# Autodesk Inventor assembly: RailWheelSys
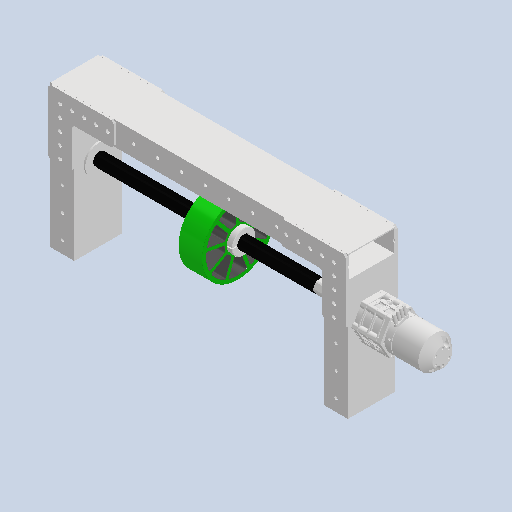
[picture p0: Inventor's stored thumbnail of the model, 512x512]
Saved by Autodesk Inventor 2022 (Build 260153000, 153)
## iProperties
Created: 2022-01-14
Part Number: RailWheelSys
Document SubType Name: Assembly
Designer: tagaz
Author: tagaz
## Documents named in this file (9)
- C:\Users\merky\OneDrive\Documents\t3-cad\CAD\2022 Parts\Index\RailWheelSys.iam
- C:\Users\merky\OneDrive\Documents\t3-cad\CAD\2022 Parts\Generic\RailSupp.ipt
- C:\Users\merky\OneDrive\Documents\t3-cad\CAD\Bearing  for THUNDER.ipt
- C:\Users\merky\OneDrive\Documents\t3-cad\CAD\2022 Parts\Generic\railThunder.ipt
- C:\Users\merky\OneDrive\Documents\t3-cad\CAD\2022 Parts\Generic\3in Compliance wheel.ipt
- C:\Users\merky\OneDrive\Documents\t3-cad\CAD\Hex Shaft Collar.ipt
- C:\Users\merky\OneDrive\Documents\t3-cad\CAD\2022 Parts\Generic\RailSupp2.ipt
- C:\Users\merky\OneDrive\Documents\t3-cad\CAD\Generic and Stock\VersaGusset 90o.ipt
- C:\Users\merky\OneDrive\Documents\t3-cad\CAD\Generic and Stock\RevMotorParts\Neo550Assembly.iam
## Components (15 placed, 8 different names)
1. RailSupp:1 — Mate:1, Flush:1, Flush:2, Insert:1, Insert:2, Mate:6, Flush:5, Mate:15, Flush:6, Flush:8, Flush:13
2. RailSupp:2 — Mate:1, Flush:1, Flush:2, Flush:10, Flush:12, Insert:3, Mate:21, Mate:22
3. Bearing  for THUNDER:1 — Insert:1
4. Bearing  for THUNDER:2 — Insert:2, Mate:2, Mate:3
5. railThunder:1 — Mate:2, Mate:3, Mate:4, Mate:5, Mate:9, Mate:10, Mate:13, Mate:14, Mate:20, Mate:24
6. 3in Compliance wheel:1 — Mate:4, Mate:5, Mate:6, Mate:11, Mate:12
7. Hex Shaft Collar:1 — Mate:9, Mate:10, Mate:11
8. Hex Shaft Collar:2 — Mate:12, Mate:13, Mate:14
9. RailSupp2:1 — Flush:5, Mate:15, Flush:6, Mate:16, Flush:7, Mate:17, Flush:9, Mate:18, Flush:11, Mate:19, Flush:14
10. VersaGusset 90o:1 — Mate:19, Flush:13, Flush:14
11. VersaGusset 90o:2 — Mate:16, Flush:7, Flush:8
12. VersaGusset 90o:3 — Mate:18, Flush:11, Flush:12
13. VersaGusset 90o:4 — Mate:17, Flush:9, Flush:10
14. Bearing  for THUNDER:3 — Insert:3, Mate:20, Mate:23
15. Neo550Assembly:1 [sub-assembly] — Mate:21, Mate:22, Mate:23, Mate:24
## Relationships (37: Mate 22, Flush 12, Insert 3)
- Mate:1 (266.7 mm): RailSupp:1 ↔ RailSupp:2
- Flush:1: RailSupp:1 ↔ RailSupp:2
- Flush:2: RailSupp:1 ↔ RailSupp:2
- Insert:1: RailSupp:1 ↔ Bearing  for THUNDER:1
- Insert:2: RailSupp:1 ↔ Bearing  for THUNDER:2
- Mate:2: Bearing  for THUNDER:2 ↔ railThunder:1
- Mate:3: Bearing  for THUNDER:2 ↔ railThunder:1
- Mate:4: railThunder:1 ↔ 3in Compliance wheel:1
- Mate:5: railThunder:1 ↔ 3in Compliance wheel:1
- Mate:6 (123.825 mm): RailSupp:1 ↔ 3in Compliance wheel:1
- Mate:9: railThunder:1 ↔ Hex Shaft Collar:1
- Mate:10: railThunder:1 ↔ Hex Shaft Collar:1
- Mate:11: 3in Compliance wheel:1 ↔ Hex Shaft Collar:1
- Mate:12: 3in Compliance wheel:1 ↔ Hex Shaft Collar:2
- Mate:13: railThunder:1 ↔ Hex Shaft Collar:2
- Mate:14: railThunder:1 ↔ Hex Shaft Collar:2
- Flush:5: RailSupp:1 ↔ RailSupp2:1
- Mate:15: RailSupp:1 ↔ RailSupp2:1
- Flush:6: RailSupp:1 ↔ RailSupp2:1
- Mate:16: RailSupp2:1 ↔ VersaGusset 90o:2
- Flush:7: RailSupp2:1 ↔ VersaGusset 90o:2
- Flush:8: RailSupp:1 ↔ VersaGusset 90o:2
- Mate:17: RailSupp2:1 ↔ VersaGusset 90o:4
- Flush:9: RailSupp2:1 ↔ VersaGusset 90o:4
- Flush:10: RailSupp:2 ↔ VersaGusset 90o:4
- Mate:18: RailSupp2:1 ↔ VersaGusset 90o:3
- Flush:11: RailSupp2:1 ↔ VersaGusset 90o:3
- Flush:12: RailSupp:2 ↔ VersaGusset 90o:3
- Mate:19: RailSupp2:1 ↔ VersaGusset 90o:1
- Flush:13: RailSupp:1 ↔ VersaGusset 90o:1
- Flush:14: RailSupp2:1 ↔ VersaGusset 90o:1
- Insert:3: RailSupp:2 ↔ Bearing  for THUNDER:3
- Mate:20: railThunder:1 ↔ Bearing  for THUNDER:3
- Mate:21: RailSupp:2 ↔ Neo550Assembly:1
- Mate:22: RailSupp:2 ↔ Neo550Assembly:1
- Mate:23: Bearing  for THUNDER:3 ↔ Neo550Assembly:1
- Mate:24: railThunder:1 ↔ Neo550Assembly:1
